# Autodesk Inventor assembly: s-assy-scara-link4
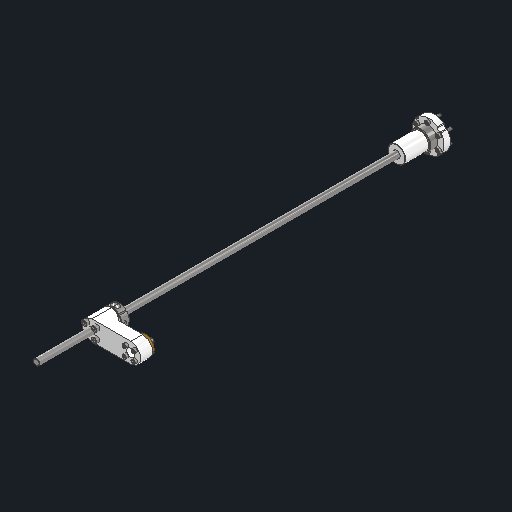
[picture p0: Inventor's stored thumbnail of the model, 512x512]
Saved by Autodesk Inventor 2022 (Build 260153000, 153)
## iProperties
Created: 2021-10-13
Part Number: s-assy-scara-link4
Document SubType Name: Assembly
Designer: Yuta Kage
Author: Yuta Kage
## Documents named in this file (12)
- C:\Users\yuta0\Documents\GitHub\catchrobo_hardware\assy-scara\s-assy-scara-link4.iam
- C:\Users\yuta0\Documents\GitHub\catchrobo_hardware\assy-scara\scara-base18.ipt
- C:\Users\yuta0\Documents\GitHub\catchrobo_hardware\assy-scara\SCSTR8-10.iam
- C:\Users\yuta0\Documents\GitHub\catchrobo_hardware\assy-scara\CB3-15.ipt
- C:\Users\yuta0\Documents\GitHub\catchrobo_hardware\assy-scara\lead-screw-nut.ipt
- C:\Users\yuta0\Documents\GitHub\catchrobo_hardware\assy-scara\scara-base17.ipt
- C:\Users\yuta0\Documents\GitHub\catchrobo_hardware\assy-scara\shaft1.ipt
- C:\Users\yuta0\Documents\GitHub\catchrobo_hardware\assy-scara\CB3-20.ipt
- C:\Users\yuta0\Documents\GitHub\catchrobo_hardware\assy-scara\LBNR3.ipt
- C:\Users\yuta0\Documents\GitHub\catchrobo_hardware\assy-scara\CB4-35.ipt
- C:\Users\yuta0\Documents\GitHub\catchrobo_hardware\assy-scara\CB4-15.ipt
- C:\Users\yuta0\Documents\GitHub\catchrobo_hardware\assy-scara\scara-base27.ipt
## Components (28 placed, 11 different names)
1. scara-base18:1 — メイト:1, メイト:2, メイト:3, メイト:7, メイト:8, メイト:9, メイト:10, メイト:19, メイト:20
2. SCSTR8-10:1 [sub-assembly] — メイト:1, メイト:2, メイト:3, メイト:11, メイト:29
3. lead-screw-nut:1 — メイト:14, メイト:15, メイト:16, メイト:26
4. scara-base17:1 — メイト:13, メイト:14, メイト:15, メイト:16, メイト:17, フラッシュ:1, フラッシュ:2, メイト:21, メイト:22, メイト:23, メイト:24, 角度:1, メイト:27
5. SCSTR8-10:2 [sub-assembly] — メイト:12, メイト:17, メイト:27
6. shaft1:1 — メイト:11, メイト:12, メイト:13, フラッシュ:1, メイト:19, メイト:28
7. scara-base27:1 — メイト:28, メイト:29
8. CB4-15:1 — メイト:7, メイト:8
9. CB4-15:2
10. CB4-15:3
11. CB3-15:1 — メイト:9, メイト:10
12. CB3-15:2
13. CB3-15:3
14. CB3-15:4
15. CB3-15:5
16. CB3-15:6
17. CB4-35:1 — メイト:21, メイト:22
18. CB4-35:2
19. CB4-35:3
20. CB4-35:4
21. CB3-20:1 — メイト:23, メイト:24, メイト:25
22. LBNR3:1 — メイト:25, メイト:26, 角度:1
23. CB3-20:2
24. LBNR3:2
25. CB3-20:3
26. LBNR3:3
27. CB3-20:4
28. LBNR3:4
## Component patterns: (3 elements, first: CB4-15:1), (6 elements, first: CB3-15:1), (4 elements, first: CB4-35:1), (4 elements, first: CB3-20:1 + LBNR3:1)
## Relationships (28: Mate 25, Flush 2, Angle 1)
- メイト:1 [Mate]: scara-base18:1 ↔ SCSTR8-10:1
- メイト:2 [Mate]: scara-base18:1 ↔ SCSTR8-10:1
- メイト:3 [Mate]: scara-base18:1 ↔ SCSTR8-10:1
- メイト:7 [Mate]: scara-base18:1 ↔ CB4-15:1
- メイト:8 [Mate]: scara-base18:1 ↔ CB4-15:1
- メイト:9 [Mate]: scara-base18:1 ↔ CB3-15:1
- メイト:10 [Mate]: scara-base18:1 ↔ CB3-15:1
- メイト:11 [Mate]: SCSTR8-10:1 ↔ shaft1:1
- メイト:12 [Mate]: SCSTR8-10:2 ↔ shaft1:1
- メイト:13 [Mate]: scara-base17:1 ↔ shaft1:1
- メイト:14 [Mate]: lead-screw-nut:1 ↔ scara-base17:1
- メイト:15 [Mate]: lead-screw-nut:1 ↔ scara-base17:1
- メイト:16 [Mate]: lead-screw-nut:1 ↔ scara-base17:1
- メイト:17 [Mate]: scara-base17:1 ↔ SCSTR8-10:2
- フラッシュ:1 [Flush] (70 mm): scara-base17:1 ↔ shaft1:1
- フラッシュ:2 [Flush]: scara-base17:1
- メイト:19 [Mate]: scara-base18:1 ↔ shaft1:1
- メイト:20 [Mate]: scara-base18:1
- メイト:21 [Mate]: scara-base17:1 ↔ CB4-35:1
- メイト:22 [Mate]: scara-base17:1 ↔ CB4-35:1
- メイト:23 [Mate]: scara-base17:1 ↔ CB3-20:1
- メイト:24 [Mate]: scara-base17:1 ↔ CB3-20:1
- メイト:25 [Mate]: CB3-20:1 ↔ LBNR3:1
- メイト:26 [Mate]: lead-screw-nut:1 ↔ LBNR3:1
- 角度:1 [Angle] (45 deg): scara-base17:1 ↔ LBNR3:1
- メイト:27 [Mate]: scara-base17:1 ↔ SCSTR8-10:2
- メイト:28 [Mate]: shaft1:1 ↔ scara-base27:1
- メイト:29 [Mate]: SCSTR8-10:1 ↔ scara-base27:1
